# Autodesk Inventor assembly: pince
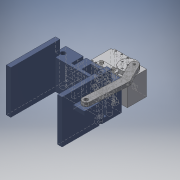
[picture p0: Inventor's stored thumbnail of the model, 180x180]
Saved by Autodesk Inventor 2017 SP1 (Build 210196100, 196)
## iProperties
Part Number: pince
Material: Générique
Document SubType Name: Assembly
Designer: Biscuit
Author: Biscuit
## Documents named in this file (5)
- C:\Users\Cortman\Google Drive\ENSEIRB\EIRBOT\COUPE 2018\Cubes\pince.iam
- C:\Users\Cortman\Google Drive\ENSEIRB\EIRBOT\COUPE 2018\Cubes\SupportPlateau.ipt
- C:\Users\Cortman\Google Drive\ENSEIRB\EIRBOT\COUPE 2018\Cubes\ax12.iam
- C:\Users\Cortman\Google Drive\ENSEIRB\EIRBOT\COUPE 2018\Cubes\membre_pince.ipt
- C:\Users\Cortman\Google Drive\ENSEIRB\EIRBOT\COUPE 2018\Cubes\bras.ipt
## Components (4 placed, 4 different names)
1. SupportPlateau:1 — Placage:4, Placage:5, Placage:6, Placage:7, Placage:8
2. ax12:1 [sub-assembly] — Placage:6, Placage:7, Placage:8, Placage:9, Placage:10
3. membre_pince:1 — Placage:4, Placage:5, Placage:11
4. bras:1 — Placage:9, Placage:10, Placage:11
## Relationships (8: Mate 8)
- Placage:4 [Mate]: SupportPlateau:1 ↔ membre_pince:1
- Placage:5 [Mate]: SupportPlateau:1 ↔ membre_pince:1
- Placage:6 [Mate]: SupportPlateau:1 ↔ ax12:1
- Placage:7 [Mate]: SupportPlateau:1 ↔ ax12:1
- Placage:8 [Mate]: SupportPlateau:1 ↔ ax12:1
- Placage:9 [Mate]: ax12:1 ↔ bras:1
- Placage:10 [Mate]: ax12:1 ↔ bras:1
- Placage:11 [Mate]: membre_pince:1 ↔ bras:1
